# Autodesk Inventor assembly: 避震器組合
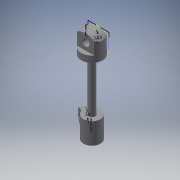
[picture p0: Inventor's stored thumbnail of the model, 180x180]
Saved by Autodesk Inventor 2019 (Build 230136000, 136)
## iProperties
Created: 2020-03-20
Part Number: 避震器組合
Material: 一般
Document SubType Name: Assembly
Designer: 黃柏維
Author: 黃柏維
## Documents named in this file (3)
- C:\機工實務\避震器組合.iam
- C:\機工實務\避震.ipt
- C:\機工實務\避震器上部.ipt
## Components (2 placed, 2 different names)
1. 避震:1 — 貼合:1
2. 避震器上部:1 — 貼合:1
## Relationships (1: Mate 1)
- 貼合:1 [Mate]: 避震:1 ↔ 避震器上部:1
